# Autodesk Inventor assembly: 520 DC Gear Motor Bracket Assembly
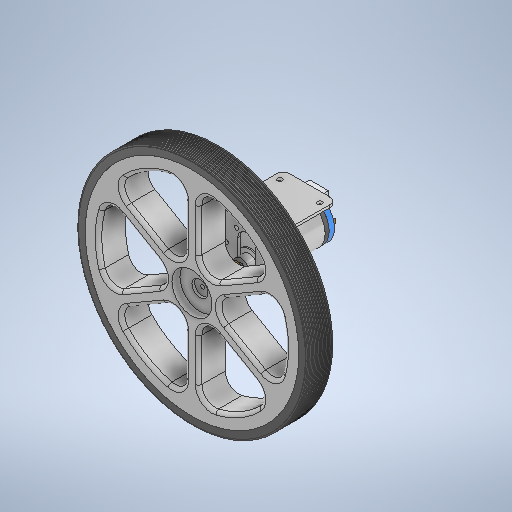
[picture p0: Inventor's stored thumbnail of the model, 512x512]
Saved by Autodesk Inventor 2025.2 (Build 292293000, 293)
## iProperties
Created: 2025-01-16
Part Number: 520 DC Gear Motor Bracket Assembly
Document SubType Name: Assembly
Designer: Matt Tidd
Author: Matt Tidd
## Documents named in this file (6)
- C:\Users\mtidd2\Desktop\H2A\CAD\Motors_and_Wheels\Wheel Assembly\Motor Wheel Assembly.iam
- C:\Users\mtidd2\Desktop\H2A\CAD\Motors_and_Wheels\520 DC Gear Motor Bracket.ipt
- C:\Users\mtidd2\Desktop\H2A\CAD\Motors_and_Wheels\520 DC Gear Motor.ipt
- C:\Users\mtidd2\Desktop\H2A\CAD\Motors_and_Wheels\Wheel Assembly\520 DC Gear Motor Wheel Coupler.ipt
- C:\Users\mtidd2\Desktop\H2A\CAD\Motors_and_Wheels\Wheel Assembly\PLA Wheel Frame.ipt
- C:\Users\mtidd2\Desktop\H2A\CAD\Motors_and_Wheels\Wheel Assembly\TPU Tire.ipt
## Components (5 placed, 5 different names)
1. 520 DC Gear Motor Wheel Coupler:1 — Mate:3, Mate:4, Mate:7
2. PLA Wheel Frame:1 — Mate:4, Mate:6, Mate:7, Mate:8
3. TPU Tire:1 — Mate:6, Mate:8
4. 520 DC Gear Motor Bracket:1 — Mate:1, Mate:2
5. 520 DC Gear Motor:1 — Mate:1, Mate:2, Mate:3
## Relationships (7: Mate 7)
- Mate:1: 520 DC Gear Motor Bracket:1 ↔ 520 DC Gear Motor:1
- Mate:2: 520 DC Gear Motor Bracket:1 ↔ 520 DC Gear Motor:1
- Mate:3: 520 DC Gear Motor Wheel Coupler:1 ↔ 520 DC Gear Motor:1
- Mate:4: 520 DC Gear Motor Wheel Coupler:1 ↔ PLA Wheel Frame:1
- Mate:6: PLA Wheel Frame:1 ↔ TPU Tire:1
- Mate:7: 520 DC Gear Motor Wheel Coupler:1 ↔ PLA Wheel Frame:1
- Mate:8: PLA Wheel Frame:1 ↔ TPU Tire:1
